# Autodesk Inventor assembly: 2X24Pins
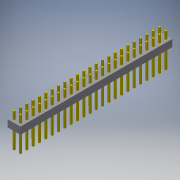
[picture p0: Inventor's stored thumbnail of the model, 180x180]
Saved by Autodesk Inventor 2019 (Build 230136000, 136)
## iProperties
Created: 2019-07-16
Part Number: 2X24Pins
Document SubType Name: Assembly
Designer: james
Author: james
## Documents named in this file (3)
- F:\JimsDesign\P1001-16bit-CPU\P1001-001 - 16bit CPU\P1001-001-210 - CAD Library\2X24Pins.iam
- F:\JimsDesign\P1001-16bit-CPU\P1001-001 - 16bit CPU\P1001-001-210 - CAD Library\1x4Pins.iam
- F:\JimsDesign\P1001-16bit-CPU\P1001-001 - 16bit CPU\P1001-001-210 - CAD Library\1x20Pins.iam
## Components (8 placed, 2 different names)
1. 1x4Pins:1 [sub-assembly] — Mate:3, Mate:4, Flush:5, Flush:6, Flush:7, Flush:8
2. 1x4Pins:2 [sub-assembly] — Mate:4, Flush:6, Flush:8, Mate:5, Flush:9, Flush:10, Flush:13
3. 1x4Pins:3 [sub-assembly] — Mate:2, Flush:3, Flush:4, Mate:3, Flush:5, Flush:7
4. 1x4Pins:4 [sub-assembly] — Mate:1, Flush:1, Flush:2
5. 1x4Pins:5 [sub-assembly] — Mate:1, Mate:2, Flush:1, Flush:2, Flush:3, Flush:4
6. 1x20Pins:1 [sub-assembly] — Mate:5, Flush:9, Flush:10, Flush:11, Flush:12, Mate:6
7. 1x4Pins:6 [sub-assembly] — Mate:7, Flush:13, Flush:14
8. 1x4Pins:7 [sub-assembly] — Flush:11, Flush:12, Mate:6, Mate:7, Flush:14
## Relationships (21: Flush 14, Mate 7)
- Mate:1: 1x4Pins:4 ↔ 1x4Pins:5
- Mate:2: 1x4Pins:3 ↔ 1x4Pins:5
- Flush:1: 1x4Pins:4 ↔ 1x4Pins:5
- Flush:2: 1x4Pins:4 ↔ 1x4Pins:5
- Flush:3: 1x4Pins:3 ↔ 1x4Pins:5
- Flush:4: 1x4Pins:3 ↔ 1x4Pins:5
- Mate:3: 1x4Pins:1 ↔ 1x4Pins:3
- Mate:4: 1x4Pins:1 ↔ 1x4Pins:2
- Flush:5: 1x4Pins:1 ↔ 1x4Pins:3
- Flush:6: 1x4Pins:1 ↔ 1x4Pins:2
- Flush:7: 1x4Pins:1 ↔ 1x4Pins:3
- Flush:8: 1x4Pins:1 ↔ 1x4Pins:2
- Mate:5: 1x4Pins:2 ↔ 1x20Pins:1
- Flush:9: 1x4Pins:2 ↔ 1x20Pins:1
- Flush:10: 1x4Pins:2 ↔ 1x20Pins:1
- Flush:11: 1x20Pins:1 ↔ 1x4Pins:7
- Flush:12: 1x20Pins:1 ↔ 1x4Pins:7
- Mate:6: 1x20Pins:1 ↔ 1x4Pins:7
- Mate:7: 1x4Pins:6 ↔ 1x4Pins:7
- Flush:13: 1x4Pins:2 ↔ 1x4Pins:6
- Flush:14: 1x4Pins:6 ↔ 1x4Pins:7
